# Autodesk Inventor assembly: Connecting Rod Assembly
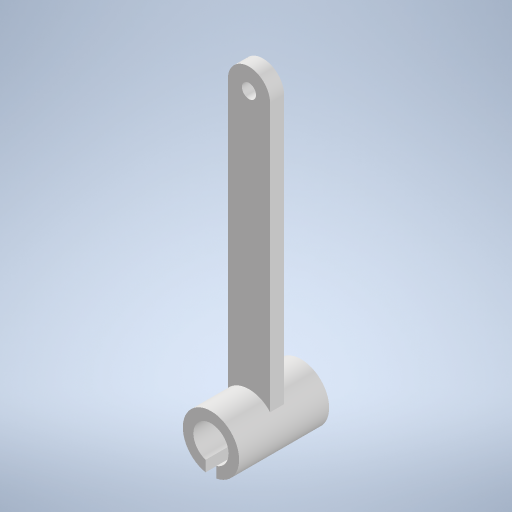
[picture p0: Inventor's stored thumbnail of the model, 512x512]
Saved by Autodesk Inventor 2023 (Build 270158000, 158)
## iProperties
Created: 2023-02-24
Part Number: Connecting Rod Assembly
Document SubType Name: Assembly
Designer: tommy
Author: tommy
## Documents named in this file (3)
- C:\Users\tommy\Documents\Repositories\Steam-Engine\Les Proper Steam Engine\CAD\Connecting Rod Assembly.iam
- C:\Users\tommy\Documents\Repositories\Steam-Engine\Les Proper Steam Engine\CAD\Conn Rod Crank Connector.ipt
- C:\Users\tommy\Documents\Repositories\Steam-Engine\Les Proper Steam Engine\CAD\Conn Rod Rod Portion.ipt
## Components (2 placed, 2 different names)
1. Conn Rod Crank Connector:1 — Angle:1, Mate:1, Flush:1
2. Conn Rod Rod Portion:1 — Angle:1, Mate:1, Flush:1
## Relationships (3: Angle 1, Mate 1, Flush 1)
- Angle:1 (0 deg): Conn Rod Crank Connector:1 ↔ Conn Rod Rod Portion:1
- Mate:1: Conn Rod Crank Connector:1 ↔ Conn Rod Rod Portion:1
- Flush:1 (2.1431 mm): Conn Rod Crank Connector:1 ↔ Conn Rod Rod Portion:1
